# Autodesk Inventor assembly: Carcaza
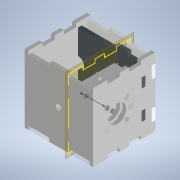
[picture p0: Inventor's stored thumbnail of the model, 180x180]
Saved by Autodesk Inventor 2020.2 (Build 242310000, 310)
## iProperties
Created: 2020-03-18
Part Number: Carcaza
Document SubType Name: Assembly
Designer: ARQ SEVILLA R
Author: ARQ SEVILLA R
## Documents named in this file (13)
- D:\Facultad Ingeniería\10° Semestre\Fundamentos de Instrumentación Biomédica\Laboratorio\Pulsómetro\Carcaza\Carcaza.iam
- D:\Facultad Ingeniería\10° Semestre\Fundamentos de Instrumentación Biomédica\Laboratorio\Pulsómetro\Carcaza\Inferior.ipt
- D:\Facultad Ingeniería\10° Semestre\Fundamentos de Instrumentación Biomédica\Laboratorio\Pulsómetro\Carcaza\Frontal.ipt
- D:\Facultad Ingeniería\10° Semestre\Fundamentos de Instrumentación Biomédica\Laboratorio\Pulsómetro\Carcaza\Lateral1.ipt
- D:\Facultad Ingeniería\10° Semestre\Fundamentos de Instrumentación Biomédica\Laboratorio\Pulsómetro\Carcaza\Lateral2.ipt
- D:\Facultad Ingeniería\10° Semestre\Fundamentos de Instrumentación Biomédica\Laboratorio\Pulsómetro\Carcaza\SoporteCircuito.ipt
- D:\Facultad Ingeniería\10° Semestre\Fundamentos de Instrumentación Biomédica\Laboratorio\Pulsómetro\Carcaza\Trasera.ipt
- D:\Facultad Ingeniería\10° Semestre\Fundamentos de Instrumentación Biomédica\Laboratorio\Pulsómetro\Carcaza\SujeciónSoportes.ipt
- D:\Facultad Ingeniería\10° Semestre\Fundamentos de Instrumentación Biomédica\Laboratorio\Pulsómetro\Carcaza\DedoSoporte.ipt
- D:\Facultad Ingeniería\10° Semestre\Fundamentos de Instrumentación Biomédica\Laboratorio\Pulsómetro\Carcaza\DedoAjuste.ipt
- D:\Facultad Ingeniería\10° Semestre\Fundamentos de Instrumentación Biomédica\Laboratorio\Pulsómetro\Carcaza\SoporteSensor.ipt
- D:\Facultad Ingeniería\10° Semestre\Fundamentos de Instrumentación Biomédica\Laboratorio\Pulsómetro\Carcaza\SoporteFotos.ipt
- D:\Facultad Ingeniería\10° Semestre\Fundamentos de Instrumentación Biomédica\Laboratorio\Pulsómetro\Carcaza\Superior.ipt
## Components (19 placed, 12 different names)
1. Inferior:1 — Mate:1, Flush:2, Mate:2, Flush:4, Flush:6, Flush:8, Flush:11, Flush:13
2. Frontal:1 — Mate:1, Flush:2, Flush:3, Flush:5, Flush:7, Flush:9, Mate:3, Flush:14, Mate:4, Mate:5, Flush:16, Mate:8, Mate:9, Flush:17, Mate:10, Mate:11, Flush:19, Mate:14, Mate:15, Mate:16, Mate:18, Mate:20, Flush:20, Mate:22, Mate:23, Mate:26, Mate:27, Flush:23
3. Lateral1:1 — Mate:2, Flush:3, Flush:4, Flush:5, Flush:10, Flush:24
4. Lateral2:1 — Flush:6, Flush:7, Flush:8, Flush:12
5. SoporteCircuito:1 — Flush:9, Flush:10, Mate:3
6. Trasera:1 — Flush:11, Flush:12, Flush:13, Flush:25
7. SujeciónSoportes:1 — Flush:14, Mate:4, Mate:5, Mate:17, Mate:19
8. SujeciónSoportes:2 — Flush:16, Mate:8, Mate:9, Mate:21, Mate:25, Mate:28
9. SujeciónSoportes:3 — Flush:17, Mate:10, Mate:11
10. SujeciónSoportes:4 — Flush:19, Mate:14, Mate:15
11. DedoSoporte:1 — Mate:18, Mate:19
12. DedoSoporte:2 — Mate:16, Mate:17
13. DedoAjuste:1 — Mate:20, Mate:21
14. SujeciónSoportes:5 — Flush:20, Mate:22, Mate:23
15. SoporteSensor:1 — Mate:25, Mate:26, Mate:31, Flush:22
16. SoporteSensor:2 — Mate:27, Mate:28, Mate:29, Mate:30, Flush:21, Mate:32, Mate:33
17. SoporteFotos:1 — Mate:29, Mate:30, Flush:21, Mate:31
18. SoporteFotos:2 — Mate:32, Flush:22, Mate:33
19. Superior:1 — Flush:23, Flush:24, Flush:25
## Relationships (50: Mate 28, Flush 22)
- Mate:1: Inferior:1 ↔ Frontal:1
- Flush:2: Inferior:1 ↔ Frontal:1
- Mate:2: Inferior:1 ↔ Lateral1:1
- Flush:3: Frontal:1 ↔ Lateral1:1
- Flush:4: Inferior:1 ↔ Lateral1:1
- Flush:5: Frontal:1 ↔ Lateral1:1
- Flush:6: Inferior:1 ↔ Lateral2:1
- Flush:7: Frontal:1 ↔ Lateral2:1
- Flush:8: Inferior:1 ↔ Lateral2:1
- Flush:9: Frontal:1 ↔ SoporteCircuito:1
- Flush:10: Lateral1:1 ↔ SoporteCircuito:1
- Mate:3: Frontal:1 ↔ SoporteCircuito:1
- Flush:11: Inferior:1 ↔ Trasera:1
- Flush:12: Lateral2:1 ↔ Trasera:1
- Flush:13: Inferior:1 ↔ Trasera:1
- Flush:14: Frontal:1 ↔ SujeciónSoportes:1
- Mate:4: Frontal:1 ↔ SujeciónSoportes:1
- Mate:5: Frontal:1 ↔ SujeciónSoportes:1
- Flush:16: Frontal:1 ↔ SujeciónSoportes:2
- Mate:8: Frontal:1 ↔ SujeciónSoportes:2
- Mate:9: Frontal:1 ↔ SujeciónSoportes:2
- Flush:17: Frontal:1 ↔ SujeciónSoportes:3
- Mate:10: Frontal:1 ↔ SujeciónSoportes:3
- Mate:11: Frontal:1 ↔ SujeciónSoportes:3
- Flush:19: Frontal:1 ↔ SujeciónSoportes:4
- Mate:14: Frontal:1 ↔ SujeciónSoportes:4
- Mate:15: Frontal:1 ↔ SujeciónSoportes:4
- Mate:16: Frontal:1 ↔ DedoSoporte:2
- Mate:17: SujeciónSoportes:1 ↔ DedoSoporte:2
- Mate:18: Frontal:1 ↔ DedoSoporte:1
- Mate:19: SujeciónSoportes:1 ↔ DedoSoporte:1
- Mate:20: Frontal:1 ↔ DedoAjuste:1
- Mate:21: SujeciónSoportes:2 ↔ DedoAjuste:1
- Flush:20: Frontal:1 ↔ SujeciónSoportes:5
- Mate:22: Frontal:1 ↔ SujeciónSoportes:5
- Mate:23: Frontal:1 ↔ SujeciónSoportes:5
- Mate:25: SujeciónSoportes:2 ↔ SoporteSensor:1
- Mate:26: Frontal:1 ↔ SoporteSensor:1
- Mate:27: Frontal:1 ↔ SoporteSensor:2
- Mate:28: SujeciónSoportes:2 ↔ SoporteSensor:2
- Mate:29: SoporteSensor:2 ↔ SoporteFotos:1
- Mate:30: SoporteSensor:2 ↔ SoporteFotos:1
- Flush:21: SoporteSensor:2 ↔ SoporteFotos:1
- Mate:31: SoporteSensor:1 ↔ SoporteFotos:1
- Mate:32: SoporteSensor:2 ↔ SoporteFotos:2
- Flush:22: SoporteSensor:1 ↔ SoporteFotos:2
- Mate:33: SoporteSensor:2 ↔ SoporteFotos:2
- Flush:23: Frontal:1 ↔ Superior:1
- Flush:24: Lateral1:1 ↔ Superior:1
- Flush:25: Trasera:1 ↔ Superior:1
